# Autodesk Inventor assembly: Ensamble
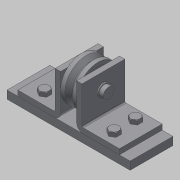
[picture p0: Inventor's stored thumbnail of the model, 180x180]
Saved by Autodesk Inventor 2019 (Build 230136000, 136)
## iProperties
Created: 2019-05-15
Part Number: Ensamble
Document SubType Name: Assembly
Designer: Gustavo Marin
Author: Gustavo Marin
## Documents named in this file (9)
- C:\Users\gusta\Documents\UPB\Diseño\Github\Activity 1\Assembly\Ensamble.iam
- C:\Users\gusta\Documents\UPB\Diseño\Github\Activity 1\Parts\Base.ipt
- C:\Users\gusta\Documents\UPB\Diseño\Github\Activity 1\Parts\Soporte.ipt
- C:\Users\gusta\Documents\UPB\Diseño\Github\Activity 1\Parts\Tornillo.ipt
- C:\Users\gusta\Documents\UPB\Diseño\Github\Activity 1\Parts\Rueda.ipt
- C:\Users\gusta\Documents\UPB\Diseño\Github\Activity 1\Parts\Washer.ipt
- C:\Users\gusta\Documents\UPB\Diseño\Github\Activity 1\Parts\Bushing.ipt
- C:\Users\gusta\Documents\UPB\Diseño\Github\Activity 1\Parts\Nut.ipt
- C:\Users\gusta\Documents\UPB\Diseño\Github\Activity 1\Parts\Bolt.ipt
## Components (13 placed, 8 different names)
1. Base:1 — Mate:1, Mate:2, Mate:3, Mate:4, Mate:5, Mate:6
2. Soporte:1 — Mate:1, Mate:2, Mate:3, Mate:7, Mate:12, Mate:13, Mate:23, Mate:24, Mate:25, Mate:26
3. Soporte:2 — Mate:4, Mate:5, Mate:6, Mate:9, Mate:16, Mate:19, Mate:20, Mate:21, Mate:22
4. Tornillo:1 — Mate:7, Mate:8, Mate:10, Mate:11, Mate:14, Mate:15, Mate:17
5. Rueda:1 — Mate:8, Mate:9
6. Washer:1 — Mate:10, Mate:13, Mate:14
7. Bushing:1 — Mate:11, Mate:12
8. Washer:2 — Mate:15, Mate:16, Mate:18
9. Nut:1 — Mate:17, Mate:18
10. Bolt:1 — Mate:19, Mate:20
11. Bolt:2 — Mate:21, Mate:22
12. Bolt:3 — Mate:23, Mate:24
13. Bolt:4 — Mate:25, Mate:26
## Relationships (26: Mate 26)
- Mate:1: Base:1 ↔ Soporte:1
- Mate:2: Base:1 ↔ Soporte:1
- Mate:3: Base:1 ↔ Soporte:1
- Mate:4: Base:1 ↔ Soporte:2
- Mate:5: Base:1 ↔ Soporte:2
- Mate:6: Base:1 ↔ Soporte:2
- Mate:7: Soporte:1 ↔ Tornillo:1
- Mate:8: Tornillo:1 ↔ Rueda:1
- Mate:9: Soporte:2 ↔ Rueda:1
- Mate:10: Tornillo:1 ↔ Washer:1
- Mate:11: Tornillo:1 ↔ Bushing:1
- Mate:12: Soporte:1 ↔ Bushing:1
- Mate:13: Soporte:1 ↔ Washer:1
- Mate:14: Tornillo:1 ↔ Washer:1
- Mate:15: Tornillo:1 ↔ Washer:2
- Mate:16: Soporte:2 ↔ Washer:2
- Mate:17: Tornillo:1 ↔ Nut:1
- Mate:18: Washer:2 ↔ Nut:1
- Mate:19: Soporte:2 ↔ Bolt:1
- Mate:20: Soporte:2 ↔ Bolt:1
- Mate:21: Soporte:2 ↔ Bolt:2
- Mate:22: Soporte:2 ↔ Bolt:2
- Mate:23: Soporte:1 ↔ Bolt:3
- Mate:24: Soporte:1 ↔ Bolt:3
- Mate:25: Soporte:1 ↔ Bolt:4
- Mate:26: Soporte:1 ↔ Bolt:4
